# Autodesk Inventor assembly: Merc2015_Assembly1
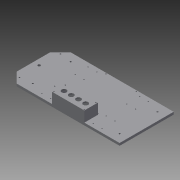
[picture p0: Inventor's stored thumbnail of the model, 180x180]
Saved by Autodesk Inventor 2015 (Build 190159000, 159)
## iProperties
Created: 2015-04-06
Part Number: Merc2015_Assembly1
Document SubType Name: Assembly
Designer: Judson
Author: Judson
## Documents named in this file (3)
- E:\Users\Judson\Documents\GitHub\CAD-Files\Mercury_2015\Merc2015_Assembly1.iam
- E:\Users\Judson\Documents\GitHub\CAD-Files\Mercury_2015\Base.ipt
- E:\Users\Judson\Documents\GitHub\CAD-Files\Mercury_2015\SwitchPanel.ipt
## Components (2 placed, 2 different names)
1. Base:1 — Mate:1, Mate:2, Mate:3, Mate:4, Mate:5
2. SwitchPanel:1 — Mate:1, Mate:2, Mate:3, Mate:4, Mate:5
## Relationships (5: Mate 5)
- Mate:1: Base:1 ↔ SwitchPanel:1
- Mate:2: Base:1 ↔ SwitchPanel:1
- Mate:3: Base:1 ↔ SwitchPanel:1
- Mate:4: Base:1 ↔ SwitchPanel:1
- Mate:5: Base:1 ↔ SwitchPanel:1
